# Autodesk Inventor assembly: Arm 2.0 Assembly
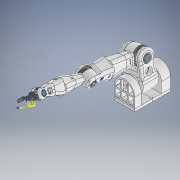
[picture p0: Inventor's stored thumbnail of the model, 180x180]
Saved by Autodesk Inventor 2017 SP1 (Build 210196100, 196)
## iProperties
Created: 2017-09-28
Part Number: Arm 2.0 Assembly
Document SubType Name: Assembly
Designer: Zach
Author: Zach
## Documents named in this file (43)
- C:\Users\Zach\Documents\GitHub\tr1\src\Body\Arm 2.0 Assembly\Arm 2.0 Assembly.iam
- C:\Users\Zach\Documents\GitHub\tr1\src\Body\Arm 2.0 Assembly\Steel Rod 8mm x 135mm.ipt
- C:\Users\Zach\Documents\GitHub\tr1\lib\22x8x8mm Bearing.ipt
- C:\Users\Zach\Documents\GitHub\tr1\src\Body\Arm 2.0 Assembly\AA004.ipt
- C:\Users\Zach\Documents\GitHub\tr1\src\Body\Arm 2.0 Assembly\AA005.ipt
- C:\Users\Zach\Documents\GitHub\tr1\src\Body\Arm 2.0 Assembly\AA006.ipt
- C:\Users\Zach\Documents\GitHub\tr1\src\Body\Arm 2.0 Assembly\AA007.ipt
- C:\Users\Zach\Documents\GitHub\tr1\lib\QS12MM250\QS12MM250.ipt
- C:\Users\Zach\Documents\GitHub\tr1\src\Body\Arm 2.0 Assembly\AA010.ipt
- C:\Users\Zach\Documents\GitHub\tr1\src\Body\Arm 2.0 Assembly\Steel Rod 8mm x 100mm.ipt
- C:\Users\Zach\Documents\GitHub\tr1\src\Body\Arm 2.0 Assembly\AA013.ipt
- C:\Users\Zach\Documents\GitHub\tr1\src\Body\Arm 2.0 Assembly\AA014.ipt
- C:\Users\Zach\Documents\GitHub\tr1\lib\12V DC Motor 378-1.ipt
- C:\Users\Zach\Documents\Inventor\Content Center Files\R2017\en-US\ISO 4016\ISO 4016 - M5 x 25.ipt
- C:\Users\Zach\Documents\Inventor\Content Center Files\R2017\en-US\ISO 4017(1)\ISO 4017 - M5 x 12 - ISO.ipt
- C:\Users\Zach\Documents\Inventor\Content Center Files\R2017\en-US\ISO 4017(1)\ISO 4017 - M5 x 20 - ISO.ipt
- C:\Users\Zach\Documents\GitHub\tr1\src\Body\Arm 2.0 Assembly\AA019.ipt
- C:\Users\Zach\Documents\GitHub\tr1\src\Body\Arm 2.0 Assembly\AA020.ipt
- C:\Users\Zach\Documents\GitHub\tr1\src\Body\Arm 2.0 Assembly\AA021.ipt
- C:\Users\Zach\Documents\GitHub\tr1\src\Body\Arm 2.0 Assembly\Steel Rod 8mm x 80mm.ipt
- C:\Users\Zach\Documents\GitHub\tr1\src\Body\Arm 2.0 Assembly\AA023.ipt
- C:\Users\Zach\Documents\GitHub\BCN3D-Moveo\Autodesk Inventor files\Gripper B Assembly.iam
- C:\Users\Zach\Documents\Inventor\Content Center Files\R2017\en-US\CNS 4320\CNS 4320 - M8 x 1 x 100.ipt
- C:\Users\Zach\Documents\GitHub\tr1\lib\AS 1110 - M8 x 150.ipt
- C:\Users\Zach\Documents\GitHub\tr1\lib\8mm Hub.ipt
- C:\Users\Zach\Documents\GitHub\tr1\src\Body\Arm 2.0 Assembly\Arm 2.0 Assembly\Design Accelerator\Spur Gears5.iam
- C:\Users\Zach\Documents\GitHub\tr1\lib\4mm mounting hub.ipt
- C:\Users\Zach\Documents\GitHub\tr1\lib\6201RS\6201RS.ipt
- C:\Users\Zach\Documents\GitHub\tr1\lib\U51105\U51105.ipt
- C:\Users\Zach\Documents\GitHub\tr1\src\Body\Arm 2.0 Assembly\AA033.ipt
- C:\Users\Zach\Documents\GitHub\tr1\src\Body\Arm 2.0 Assembly\AA032.ipt
- C:\Users\Zach\Documents\GitHub\tr1\src\Body\Arm 2.0 Assembly\AA031.ipt
- C:\Users\Zach\Documents\GitHub\tr1\lib\Timing Pulley - T5 4mm Bore 15mm Width.ipt
- C:\Users\Zach\Documents\GitHub\tr1\src\Body\Arm 2.0 Assembly\AA034.ipt
- C:\Users\Zach\Documents\GitHub\tr1\src\Body\Arm 2.0 Assembly\Arm 2.0 Assembly\Design Accelerator\Spur Gears6.iam
- C:\Users\Zach\Documents\GitHub\tr1\src\Body\Arm 2.0 Assembly\AA001b.ipt
- C:\Users\Zach\Documents\GitHub\tr1\src\Body\Arm 2.0 Assembly\AA008c.ipt
- C:\Users\Zach\Documents\GitHub\tr1\src\Body\Arm 2.0 Assembly\AA008d.ipt
- C:\Users\Zach\Documents\GitHub\tr1\src\Body\Arm 2.0 Assembly\AA035.ipt
- C:\Users\Zach\Documents\GitHub\tr1\src\Body\Arm 2.0 Assembly\Arm 2.0 Assembly\Design Accelerator\Spur Gears7.iam
- C:\Users\Zach\Documents\GitHub\tr1\src\Body\Arm 2.0 Assembly\AA036.ipt
- C:\Users\Zach\Documents\GitHub\tr1\src\Body\Arm 2.0 Assembly\AA037.ipt
- C:\Users\Zach\Documents\GitHub\tr1\src\Body\Arm 2.0 Assembly\AA016b.ipt
## Components (80 placed, 40 different names)
1. AA001b:1 — Mate:414, Mate:415, Mate:416, Mate:421, Mate:422, Mate:423, Mate:431, Mate:432, Flush:18, Flush:19, Mate:434, Mate:435, Flush:20, Mate:438, Mate:439, Mate:440, Mate:443, Mate:444, Mate:445
2. AA004:1 — Mate:23, Mate:345, Mate:347, Mate:350, Mate:352, Mate:353, Mate:357, Mate:414, Mate:431, Mate:435
3. AA005:1 — Mate:99, Mate:100, Mate:103, Mate:331, Mate:332, Mate:333, Mate:341, Mate:381
4. AA006:1 — Mate:24, Mate:25, Mate:96, Mate:97, Mate:98, Mate:382, Mate:383, Mate:485
5. AA007:1 — Mate:19, Mate:20, Mate:99, Mate:100, Mate:103, Mate:483
6. AA007:2 — Mate:19, Mate:20, Mate:96, Mate:97, Mate:98
7. AA008c:1 — Mate:449, Mate:450, Mate:451, Mate:452, Mate:453, Mate:454, Mate:463, Mate:464, Mate:466, Mate:467, Mate:481, Mate:497
8. AA008d:1 — Mate:455, Mate:456, Mate:457, Mate:461, Mate:463, Mate:464, Mate:466, Mate:467, Mate:480, Mate:482
9. AA010:1 — Mate:55, Flush:6, Mate:56, Flush:7, Flush:8, Mate:64, Mate:65, Mate:66, Mate:67, Mate:68, Mate:69, Mate:486, Mate:487, Mate:488, Mate:490, Mate:492, Mate:493, Mate:494, Mate:495, Mate:496, Mate:497
10. AA013:1 — Mate:148, Mate:149, Mate:150, Mate:151, Mate:152, Mate:153, Mate:434, Mate:436
11. AA013:2 — Mate:142, Mate:143, Mate:144, Mate:145, Mate:146, Mate:147, Mate:439
12. AA014:1 — Mate:64, Mate:65, Mate:66, Mate:160, Mate:161, Mate:162, Mate:163, Mate:164, Mate:165
13. AA014:2 — Mate:67, Mate:68, Mate:69, Mate:154, Mate:155, Mate:156, Mate:157, Mate:158, Mate:159
14. AA016b:1 — Mate:518, Mate:519, Mate:520, Mate:521, Mate:525, Mate:526, Mate:527, Mate:529, Mate:530
15. AA019:1 — Mate:174, Mate:175, Mate:182, Mate:183, Mate:185, Flush:15, Flush:16, Flush:17, Mate:188, Mate:189, Mate:190, Mate:191, Mate:192, Mate:193, Mate:388, Mate:400, Mate:401, Mate:533, Mate:536
16. AA020:1 — Mate:171, Mate:172, Mate:173, Mate:175, Mate:194, Mate:196
17. AA021:1 — Mate:171, Mate:172, Mate:173, Mate:174, Mate:195
18. AA023:1 — Mate:188, Mate:189, Mate:193
19. AA023:2 — Mate:190, Mate:191, Mate:192
20. AA031:1 — Mate:366, Mate:367, Mate:523, Mate:524
21. AA032:2 — Mate:465
22. AA033:1 — Mate:351, Mate:352, Mate:353, Mate:355, Mate:356
23. AA034:1 — Mate:388, Mate:529, Mate:533, Mate:534, Mate:535, Mate:536
24. AA036:1 — Mate:498, Mate:500, Mate:501, Mate:502, Mate:503, Mate:511
25. AA037:1 — Mate:501, Mate:502, Mate:503, Mate:514, Mate:515, Mate:516, Mate:517, Mate:518, Mate:519, Mate:520, Mate:530
26. Gripper B Assembly:1 [sub-assembly] — Mate:194, Mate:195, Mate:196
27. 22x8x8mm Bearing:1 — Mate:433, Flush:18
28. 22x8x8mm Bearing:2 — Mate:437, Flush:20
29. 22x8x8mm Bearing:3 — Mate:55, Flush:6, Mate:57
30. 22x8x8mm Bearing:4 — Mate:56, Flush:7
31. 22x8x8mm Bearing:5 — Mate:186, Flush:16
32. 22x8x8mm Bearing:6 — Mate:187, Flush:17
33. 22x8x8mm Bearing:7 — Mate:264, Mate:526
34. 22x8x8mm Bearing:8 — Mate:527, Mate:528
35. 22x8x8mm Bearing:13 — Mate:451, Mate:452
36. 22x8x8mm Bearing:14 — Mate:449, Mate:450
37. QS12MM250:1 — Mate:23, Mate:24, Mate:25, Mate:344, Mate:346, Mate:348, Mate:351, Mate:354, Mate:484
38. Steel Rod 8mm x 135mm:1 — Mate:432, Mate:433, Flush:19, Mate:436, Mate:437, Mate:476, Mate:477
39. Steel Rod 8mm x 100mm:1 — Mate:57, Flush:8, Mate:491, Mate:498
40. Steel Rod 8mm x 80mm:1 — Mate:185, Flush:15, Mate:186, Mate:187
41. 12V DC Motor 378-1:1 — Mate:371, Mate:421, Mate:422, Mate:423, Mate:474
42. 12V DC Motor 378-1:2 — Mate:376, Mate:486, Mate:487, Mate:488, Mate:489
43. 12V DC Motor 378-1:3 — Mate:182, Mate:183, Mate:392, Mate:394, Mate:400
44. 12V DC Motor 378-1:4 — Mate:514, Mate:515, Mate:516, Mate:522
45. 12V DC Motor 378-1:6 — Mate:331, Mate:332, Mate:333, Mate:340, Mate:342
46. 12V DC Motor 378-1:7 — Mate:455, Mate:456, Mate:457, Mate:460, Mate:465
47. 6201RS:1 — Mate:346, Mate:347
48. 6201RS:2 — Mate:356, Mate:357
49. U51105:1 — Mate:348, Mate:349, Mate:381
50. U51105:2 — Mate:354, Mate:355, Mate:382, Mate:383
51. 8mm Hub:1
52. 8mm Hub:2 — Mate:368, Mate:531, Mate:534, Mate:535
53. 8mm Hub:3 — Mate:493, Mate:494, Mate:495
54. 4mm mounting hub:1 — Mate:340, Mate:341, Mate:343
55. 4mm mounting hub:3 — Mate:366, Mate:367, Mate:517, Mate:522, Mate:523, Mate:524
56. 4mm mounting hub:4 — Mate:371, Mate:443
57. 4mm mounting hub:5 — Mate:376, Mate:513
58. 4mm mounting hub:6 — Mate:392, Mate:395, Mate:396, Mate:401
59. 4mm mounting hub:7 — Mate:460, Mate:461
60. Timing Pulley - T5 4mm Bore 15mm Width:3 — Mate:394, Mate:395, Mate:396
61. ISO 4016 M5 x 25:9 — Mate:415
62. ISO 4016 M5 x 25:10 — Mate:416
63. ISO 4017 M5 x 20:1 — Mate:146, Mate:147, Mate:438
64. ISO 4017 M5 x 20:2 — Mate:144, Mate:145, Mate:440
65. ISO 4017 M5 x 20:3 — Mate:142, Mate:143
66. ISO 4017 M5 x 20:4 — Mate:148, Mate:149
67. ISO 4017 M5 x 20:5 — Mate:152, Mate:153
68. ISO 4017 M5 x 20:6 — Mate:150, Mate:151
69. ISO 4017 M5 x 12:1 — Mate:154, Mate:155
70. ISO 4017 M5 x 12:2 — Mate:156, Mate:158
71. ISO 4017 M5 x 12:3 — Mate:157, Mate:159
72. ISO 4017 M5 x 12:4 — Mate:160, Mate:161
73. ISO 4017 M5 x 12:5 — Mate:162, Mate:163
74. ISO 4017 M5 x 12:6 — Mate:164, Mate:165
75. CNS 4320 M8 x 100:1 — Mate:264, Mate:368, Mate:521, Mate:525, Mate:528, Mate:531
76. AS 1110 - Metric M8 x 80:2 — Mate:453, Mate:454, Mate:496
77. Spur Gears:5 [sub-assembly] — Mate:342, Mate:343, Mate:344, Mate:345, Mate:349, Mate:350
78. Spur Gears:6 [sub-assembly] — Mate:444, Mate:445, Mate:474, Mate:476, Mate:478, Mate:479
79. Spur Gear2:1 — Mate:477, Mate:478, Mate:479, Mate:480, Mate:481, Mate:482
80. Spur Gears:7 [sub-assembly] — Mate:489, Mate:490, Mate:491, Mate:492, Mate:500, Mate:511, Mate:513
## Relationships (198: Mate 189, Flush 9)
- Mate:19: AA007:1 ↔ AA007:2
- Mate:20: AA007:1 ↔ AA007:2
- Mate:23: AA004:1 ↔ QS12MM250:1
- Mate:24: AA006:1 ↔ QS12MM250:1
- Mate:25: AA006:1 ↔ QS12MM250:1
- Mate:55: AA010:1 ↔ 22x8x8mm Bearing:3
- Flush:6: AA010:1 ↔ 22x8x8mm Bearing:3
- Mate:56: AA010:1 ↔ 22x8x8mm Bearing:4
- Flush:7: AA010:1 ↔ 22x8x8mm Bearing:4
- Mate:57: 22x8x8mm Bearing:3 ↔ Steel Rod 8mm x 100mm:1
- Flush:8 (2.5 mm): AA010:1 ↔ Steel Rod 8mm x 100mm:1
- Mate:64: AA010:1 ↔ AA014:1
- Mate:65: AA010:1 ↔ AA014:1
- Mate:66: AA010:1 ↔ AA014:1
- Mate:67: AA010:1 ↔ AA014:2
- Mate:68: AA010:1 ↔ AA014:2
- Mate:69: AA010:1 ↔ AA014:2
- Mate:96: AA006:1 ↔ AA007:2
- Mate:97: AA006:1 ↔ AA007:2
- Mate:98: AA006:1 ↔ AA007:2
- Mate:99: AA005:1 ↔ AA007:1
- Mate:100: AA005:1 ↔ AA007:1
- Mate:103: AA005:1 ↔ AA007:1
- Mate:142: AA013:2 ↔ ISO 4017 M5 x 20:3
- Mate:143: AA013:2 ↔ ISO 4017 M5 x 20:3
- Mate:144: AA013:2 ↔ ISO 4017 M5 x 20:2
- Mate:145: AA013:2 ↔ ISO 4017 M5 x 20:2
- Mate:146: AA013:2 ↔ ISO 4017 M5 x 20:1
- Mate:147: AA013:2 ↔ ISO 4017 M5 x 20:1
- Mate:148: AA013:1 ↔ ISO 4017 M5 x 20:4
- Mate:149: AA013:1 ↔ ISO 4017 M5 x 20:4
- Mate:150: AA013:1 ↔ ISO 4017 M5 x 20:6
- Mate:151: AA013:1 ↔ ISO 4017 M5 x 20:6
- Mate:152: AA013:1 ↔ ISO 4017 M5 x 20:5
- Mate:153: AA013:1 ↔ ISO 4017 M5 x 20:5
- Mate:154: AA014:2 ↔ ISO 4017 M5 x 12:1
- Mate:155: AA014:2 ↔ ISO 4017 M5 x 12:1
- Mate:156: AA014:2 ↔ ISO 4017 M5 x 12:2
- Mate:157: AA014:2 ↔ ISO 4017 M5 x 12:3
- Mate:158: AA014:2 ↔ ISO 4017 M5 x 12:2
- Mate:159: AA014:2 ↔ ISO 4017 M5 x 12:3
- Mate:160: AA014:1 ↔ ISO 4017 M5 x 12:4
- Mate:161: AA014:1 ↔ ISO 4017 M5 x 12:4
- Mate:162: AA014:1 ↔ ISO 4017 M5 x 12:5
- Mate:163: AA014:1 ↔ ISO 4017 M5 x 12:5
- Mate:164: AA014:1 ↔ ISO 4017 M5 x 12:6
- Mate:165: AA014:1 ↔ ISO 4017 M5 x 12:6
- Mate:171: AA020:1 ↔ AA021:1
- Mate:172: AA020:1 ↔ AA021:1
- Mate:173: AA020:1 ↔ AA021:1
- Mate:174 (1 mm): AA019:1 ↔ AA021:1
- Mate:175: AA019:1 ↔ AA020:1
- Mate:182: AA019:1 ↔ 12V DC Motor 378-1:3
- Mate:183: AA019:1 ↔ 12V DC Motor 378-1:3
- Mate:185: AA019:1 ↔ Steel Rod 8mm x 80mm:1
- Flush:15: AA019:1 ↔ Steel Rod 8mm x 80mm:1
- Mate:186: 22x8x8mm Bearing:5 ↔ Steel Rod 8mm x 80mm:1
- Flush:16: AA019:1 ↔ 22x8x8mm Bearing:5
- Mate:187: 22x8x8mm Bearing:6 ↔ Steel Rod 8mm x 80mm:1
- Flush:17: AA019:1 ↔ 22x8x8mm Bearing:6
- Mate:188: AA019:1 ↔ AA023:1
- Mate:189: AA019:1 ↔ AA023:1
- Mate:190: AA019:1 ↔ AA023:2
- Mate:191: AA019:1 ↔ AA023:2
- Mate:192: AA019:1 ↔ AA023:2
- Mate:193: AA019:1 ↔ AA023:1
- Mate:194: AA020:1 ↔ Gripper B Assembly:1
- Mate:195: AA021:1 ↔ Gripper B Assembly:1
- Mate:196: AA020:1 ↔ Gripper B Assembly:1
- Mate:264: 22x8x8mm Bearing:7 ↔ CNS 4320 M8 x 100:1
- Mate:331: AA005:1 ↔ 12V DC Motor 378-1:6
- Mate:332: AA005:1 ↔ 12V DC Motor 378-1:6
- Mate:333: AA005:1 ↔ 12V DC Motor 378-1:6
- Mate:340: 12V DC Motor 378-1:6 ↔ 4mm mounting hub:1
- Mate:341: AA005:1 ↔ 4mm mounting hub:1
- Mate:342: 12V DC Motor 378-1:6 ↔ Spur Gears:5
- Mate:343: 4mm mounting hub:1 ↔ Spur Gears:5
- Mate:344: QS12MM250:1 ↔ Spur Gears:5
- Mate:345: AA004:1 ↔ Spur Gears:5
- Mate:346: QS12MM250:1 ↔ 6201RS:1
- Mate:347: AA004:1 ↔ 6201RS:1
- Mate:348: QS12MM250:1 ↔ U51105:1
- Mate:349: U51105:1 ↔ Spur Gears:5
- Mate:350: AA004:1 ↔ Spur Gears:5
- Mate:351: AA033:1 ↔ QS12MM250:1
- Mate:352: AA004:1 ↔ AA033:1
- Mate:353: AA004:1 ↔ AA033:1
- Mate:354: QS12MM250:1 ↔ U51105:2
- Mate:355: AA033:1 ↔ U51105:2
- Mate:356: AA033:1 ↔ 6201RS:2
- Mate:357: AA004:1 ↔ 6201RS:2
- Mate:366: AA031:1 ↔ 4mm mounting hub:3
- Mate:367: AA031:1 ↔ 4mm mounting hub:3
- Mate:368: 8mm Hub:2 ↔ CNS 4320 M8 x 100:1
- Mate:371: 12V DC Motor 378-1:1 ↔ 4mm mounting hub:4
- Mate:376: 12V DC Motor 378-1:2 ↔ 4mm mounting hub:5
- Mate:381 (1 mm): AA005:1 ↔ U51105:1
- Mate:382: AA006:1 ↔ U51105:2
- Mate:383: AA006:1 ↔ U51105:2
- Mate:388: AA019:1 ↔ AA034:1
- Mate:392: 12V DC Motor 378-1:3 ↔ 4mm mounting hub:6
- Mate:394: 12V DC Motor 378-1:3 ↔ Timing Pulley - T5 4mm Bore 15mm Width:3
- Mate:395: 4mm mounting hub:6 ↔ Timing Pulley - T5 4mm Bore 15mm Width:3
- Mate:396: 4mm mounting hub:6 ↔ Timing Pulley - T5 4mm Bore 15mm Width:3
- Mate:400: AA019:1 ↔ 12V DC Motor 378-1:3
- Mate:401: AA019:1 ↔ 4mm mounting hub:6
- Mate:414: AA001b:1 ↔ AA004:1
- Mate:415: AA001b:1 ↔ ISO 4016 M5 x 25:9
- Mate:416: AA001b:1 ↔ ISO 4016 M5 x 25:10
- Mate:421: AA001b:1 ↔ 12V DC Motor 378-1:1
- Mate:422: AA001b:1 ↔ 12V DC Motor 378-1:1
- Mate:423: AA001b:1 ↔ 12V DC Motor 378-1:1
- Mate:431: AA001b:1 ↔ AA004:1
- Mate:432: AA001b:1 ↔ Steel Rod 8mm x 135mm:1
- Mate:433: 22x8x8mm Bearing:1 ↔ Steel Rod 8mm x 135mm:1
- Flush:18: AA001b:1 ↔ 22x8x8mm Bearing:1
- Flush:19 (-2.5 mm): AA001b:1 ↔ Steel Rod 8mm x 135mm:1
- Mate:434: AA001b:1 ↔ AA013:1
- Mate:435: AA001b:1 ↔ AA004:1
- Mate:436: AA013:1 ↔ Steel Rod 8mm x 135mm:1
- Mate:437: 22x8x8mm Bearing:2 ↔ Steel Rod 8mm x 135mm:1
- Flush:20: AA001b:1 ↔ 22x8x8mm Bearing:2
- Mate:438: AA001b:1 ↔ ISO 4017 M5 x 20:1
- Mate:439: AA001b:1 ↔ AA013:2
- Mate:440: AA001b:1 ↔ ISO 4017 M5 x 20:2
- Mate:443 (1.625 mm): AA001b:1 ↔ 4mm mounting hub:4
- Mate:444 (1.625 mm): AA001b:1 ↔ Spur Gears:6
- Mate:445 (1.625 mm): AA001b:1 ↔ Spur Gears:6
- Mate:449: AA008c:1 ↔ 22x8x8mm Bearing:14
- Mate:450: AA008c:1 ↔ 22x8x8mm Bearing:14
- Mate:451: AA008c:1 ↔ 22x8x8mm Bearing:13
- Mate:452: AA008c:1 ↔ 22x8x8mm Bearing:13
- Mate:453: AA008c:1 ↔ AS 1110 - Metric M8 x 80:2
- Mate:454: AA008c:1 ↔ AS 1110 - Metric M8 x 80:2
- Mate:455: AA008d:1 ↔ 12V DC Motor 378-1:7
- Mate:456: AA008d:1 ↔ 12V DC Motor 378-1:7
- Mate:457: AA008d:1 ↔ 12V DC Motor 378-1:7
- [Mate]: AA032:2 ↔ 4mm mounting hub:7
- [Mate]: AA032:2 ↔ 4mm mounting hub:7
- Mate:460: 12V DC Motor 378-1:7 ↔ 4mm mounting hub:7
- Mate:461: AA008d:1 ↔ 4mm mounting hub:7
- Mate:463: AA008c:1 ↔ AA008d:1
- Mate:464: AA008c:1 ↔ AA008d:1
- Mate:465: AA032:2 ↔ 12V DC Motor 378-1:7
- Mate:466: AA008c:1 ↔ AA008d:1
- Mate:467: AA008c:1 ↔ AA008d:1
- Mate:474: 12V DC Motor 378-1:1 ↔ Spur Gears:6
- Mate:476: Steel Rod 8mm x 135mm:1 ↔ Spur Gears:6
- Mate:477: Steel Rod 8mm x 135mm:1 ↔ Spur Gear2:1
- Mate:478: Spur Gears:6 ↔ Spur Gear2:1
- Mate:479: Spur Gears:6 ↔ Spur Gear2:1
- Mate:480: AA008d:1 ↔ Spur Gear2:1
- Mate:481: AA008c:1 ↔ Spur Gear2:1
- Mate:482: AA008d:1 ↔ Spur Gear2:1
- Mate:483: AA007:1
- Mate:484: QS12MM250:1
- Mate:485: AA006:1
- Mate:486: AA010:1 ↔ 12V DC Motor 378-1:2
- Mate:487: AA010:1 ↔ 12V DC Motor 378-1:2
- Mate:488: AA010:1 ↔ 12V DC Motor 378-1:2
- Mate:489: 12V DC Motor 378-1:2 ↔ Spur Gears:7
- Mate:490: AA010:1 ↔ Spur Gears:7
- Mate:491: Steel Rod 8mm x 100mm:1 ↔ Spur Gears:7
- Mate:492: AA010:1 ↔ Spur Gears:7
- Mate:493: AA010:1 ↔ 8mm Hub:3
- Mate:494: AA010:1 ↔ 8mm Hub:3
- Mate:495: AA010:1 ↔ 8mm Hub:3
- Mate:496: AA010:1 ↔ AS 1110 - Metric M8 x 80:2
- Mate:497: AA008c:1 ↔ AA010:1
- Mate:498: AA036:1 ↔ Steel Rod 8mm x 100mm:1
- Mate:500: AA036:1 ↔ Spur Gears:7
- Mate:501: AA036:1 ↔ AA037:1
- Mate:502: AA036:1 ↔ AA037:1
- Mate:503: AA036:1 ↔ AA037:1
- Mate:511: AA036:1 ↔ Spur Gears:7
- Mate:513: 4mm mounting hub:5 ↔ Spur Gears:7
- Mate:514: AA037:1 ↔ 12V DC Motor 378-1:4
- Mate:515: AA037:1 ↔ 12V DC Motor 378-1:4
- Mate:516: AA037:1 ↔ 12V DC Motor 378-1:4
- Mate:517: AA037:1 ↔ 4mm mounting hub:3
- Mate:518: AA016b:1 ↔ AA037:1
- Mate:519: AA016b:1 ↔ AA037:1
- Mate:520: AA016b:1 ↔ AA037:1
- Mate:521: AA016b:1 ↔ CNS 4320 M8 x 100:1
- Mate:522: 12V DC Motor 378-1:4 ↔ 4mm mounting hub:3
- Mate:523: AA031:1 ↔ 4mm mounting hub:3
- Mate:524: AA031:1 ↔ 4mm mounting hub:3
- Mate:525: AA016b:1 ↔ CNS 4320 M8 x 100:1
- Mate:526 (0.5 mm): AA016b:1 ↔ 22x8x8mm Bearing:7
- Mate:527 (0.5 mm): AA016b:1 ↔ 22x8x8mm Bearing:8
- Mate:528: 22x8x8mm Bearing:8 ↔ CNS 4320 M8 x 100:1
- Mate:529: AA016b:1 ↔ AA034:1
- Mate:530: AA016b:1 ↔ AA037:1
- Mate:531: 8mm Hub:2 ↔ CNS 4320 M8 x 100:1
- Mate:533: AA019:1 ↔ AA034:1
- Mate:534: AA034:1 ↔ 8mm Hub:2
- Mate:535: AA034:1 ↔ 8mm Hub:2
- Mate:536: AA019:1 ↔ AA034:1
## Named parameters: d576_d462 = 0 mm, d577_d463 = 0 mm
